# Autodesk Inventor assembly: target_plate
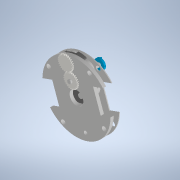
[picture p0: Inventor's stored thumbnail of the model, 180x180]
Saved by Autodesk Inventor 2021 (Build 250183000, 183)
## iProperties
Created: 2024-02-12
Part Number: target_plate
Document SubType Name: Assembly
Designer: Sebastián
Author: Sebastián
## Documents named in this file (7)
- C:\Users\Sebastián\Documents\Inventor\PLD SAP\target_plate.iam
- C:\Users\Sebastián\Documents\Inventor\PLD SAP\placa_base.ipt
- C:\Users\Sebastián\Documents\Inventor\PLD SAP\10d_coupler.ipt
- C:\Users\Sebastián\Documents\Inventor\PLD SAP\portablancos_comp.iam
- C:\Users\Sebastián\Documents\Inventor\PLD SAP\shaft_1.ipt
- C:\Users\Sebastián\Documents\Inventor\PLD SAP\cubre_blancos.ipt
- C:\Users\Sebastián\Documents\Inventor\PLD SAP\placa_blancos\Design Accelerator\Spur Gears2.iam
## Components (6 placed, 6 different names)
1. placa_base:1 — Cylindrical:2, Cylindrical:3, Angle:1, Mate:3, Mate:5
2. 10d_coupler:1 — Rotational:1
3. portablancos_comp:1 [sub-assembly] — Cylindrical:1, Mate:1, Mate:4
4. shaft_1:1 — Rotational:1, Cylindrical:1, Cylindrical:2, Mate:2
5. cubre_blancos:1 — Cylindrical:3, Angle:1, Mate:1
6. Spur Gears:1 [sub-assembly] — Mate:2, Mate:3, Mate:4, Mate:5
## Relationships (10: Mate 5, CylindricalJoint 3, RevoluteJoint 1, Angle 1)
- Rotational:1 [RevoluteJoint]: 10d_coupler:1 ↔ shaft_1:1
- Cylindrical:1: portablancos_comp:1 ↔ shaft_1:1
- Cylindrical:2: placa_base:1 ↔ shaft_1:1
- Cylindrical:3: placa_base:1 ↔ cubre_blancos:1
- Angle:1 (0 deg): placa_base:1 ↔ cubre_blancos:1
- Mate:1 (1 mm): portablancos_comp:1 ↔ cubre_blancos:1
- Mate:2: shaft_1:1 ↔ Spur Gears:1
- Mate:3: placa_base:1 ↔ Spur Gears:1
- Mate:4: portablancos_comp:1 ↔ Spur Gears:1
- Mate:5: placa_base:1 ↔ Spur Gears:1
